# Autodesk Inventor assembly: AX-12A
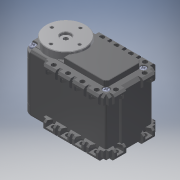
[picture p0: Inventor's stored thumbnail of the model, 180x180]
Saved by Autodesk Inventor 2019 (Build 230136000, 136)
## iProperties
Created: 2011-11-04
Part Number: AX-12A
Document SubType Name: Assembly
Designer: zreik
Sending System: SolidWorks 2012
Last Author: Dangtq
Last Saved: 2011-11-08
Author: zreik
## Documents named in this file (6)
- D:\Documents\HIAST\4th year\4th Year Project\Design\AX-12A\AX-12A.iam
- D:\Documents\HIAST\4th year\4th Year Project\Design\AX-12A\AX-12A-01.ipt
- D:\Documents\HIAST\4th year\4th Year Project\Design\AX-12A\AX-12A-02.ipt
- D:\Documents\HIAST\4th year\4th Year Project\Design\AX-12A\AX-12A-03.ipt
- D:\Documents\HIAST\4th year\4th Year Project\Design\AX-12A\AX-12A-04.ipt
- D:\Documents\HIAST\4th year\4th Year Project\Design\AX-12A\SetScrew.ipt
## Components (8 placed, 5 different names)
1. AX-12A-01:1
2. AX-12A-02:1 — Mate:1, Mate:2
3. AX-12A-03:1
4. AX-12A-04:1 — Mate:1, Mate:2
5. SetScrew:5
6. SetScrew:6
7. SetScrew:7
8. SetScrew:8
## Relationships (2: Mate 2)
- Mate:1: AX-12A-02:1 ↔ AX-12A-04:1
- Mate:2: AX-12A-02:1 ↔ AX-12A-04:1
